# Autodesk Inventor assembly: m5x6 assembly
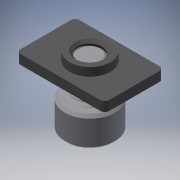
[picture p0: Inventor's stored thumbnail of the model, 180x180]
Saved by Autodesk Inventor 2016 (Build 200138000, 138)
## iProperties
Created: 2016-07-25
Part Number: m5x6 assembly
Document SubType Name: Assembly
Designer: Jonathan
Author: Jonathan
## Documents named in this file (3)
- C:\Users\Jonathan\Desktop\Models\Four Paddle Detector\frame\brackets\m5x6 assembly.iam
- C:\Users\Jonathan\Desktop\Models\Four Paddle Detector\frame\brackets\m5TNut.ipt
- C:\Users\Jonathan\Desktop\Models\Four Paddle Detector\frame\brackets\m5x6.ipt
## Components (2 placed, 2 different names)
1. m5TNut:1 — Mate:1, Mate:2
2. m5x6:1 — Mate:1, Mate:2
## Relationships (2: Mate 2)
- Mate:1: m5TNut:1 ↔ m5x6:1
- Mate:2 (3.5875 mm): m5TNut:1 ↔ m5x6:1
